# Autodesk Inventor assembly: GA_bilen
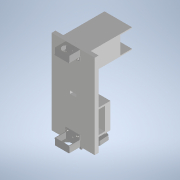
[picture p0: Inventor's stored thumbnail of the model, 180x180]
Saved by Autodesk Inventor 2022.1 (Build 261234020, 234B)
## iProperties
Created: 2022-01-29
Part Number: GA_bilen
Document SubType Name: Assembly
Designer: 46734
Author: 46734
## Documents named in this file (14)
- G:\Min enhet\GA\3d print\GA_bilen.iam
- G:\Min enhet\GA\3d print\Assembly1.iam
- G:\Min enhet\GA\3d print\body.ipt
- G:\Min enhet\GA\3d print\KameraFront v1.ipt
- G:\Min enhet\GA\3d print\poerbankhållare.ipt
- G:\Min enhet\GA\3d print\test hålare.ipt
- G:\Min enhet\GA\3d print\ULTRALJUD GA v2.ipt
- G:\Min enhet\GA\3d print\pir sensor v1.ipt
- G:\Min enhet\GA\3d print\kameraGa Langst ner v1.ipt
- G:\Min enhet\GA\3d print\rpi case 4.ipt
- C:\Users\46734\Documents\Inventor\Content Center Files\R2022\en-US\AS 1420\AS 1420 - 1973 - M3 x 10.ipt
- C:\Users\46734\Documents\Inventor\Content Center Files\R2022\en-US\ANSI B18.3.1M(1)\ANSI B18.3.1M - M2x0,4 x 10(2).ipt
- C:\Users\46734\Documents\Inventor\Content Center Files\R2022\en-US\AS 1420\AS 1420 - 1973 - M4 x 25.ipt
- C:\Users\46734\Documents\Inventor\Content Center Files\R2022\en-US\ANSI B18.2.4.2M\ANSI B18.2.4.2M - M4x0,7 - 7.ipt
## Components (24 placed, 13 different names)
1. Assembly1:1 [sub-assembly] — Mate:1, Flush:1, Flush:2, Insert:1
2. body:1 — Mate:2, Flush:3, Flush:4, Mate:3, Flush:5, Flush:6, Mate:4, Flush:7, Mate:5, Flush:9, Flush:10, Mate:10, Flush:19, Flush:20
3. KameraFront v1:1 — Mate:1, Flush:1, Flush:2
4. poerbankhållare:1 — Mate:2, Flush:3, Flush:4, Rotational:7, Rotational:8, Rotational:9, Rotational:10
5. test hålare:1 — Insert:1, Flush:17, Flush:18, Mate:9, Flush:22, Rotational:11, Rotational:12, Rigid:1, Rotational:13
6. ULTRALJUD GA v2:1 — Mate:5, Flush:9, Flush:10, Rotational:1, Rotational:2
7. pir sensor v1:1 — Mate:4, Flush:7, Flush:8, Rotational:3, Rotational:4
8. pir sensor v1:2 — Mate:3, Flush:5, Flush:6, Flush:8, Rotational:5, Rotational:6
9. kameraGa Langst ner v1:1 — Flush:17, Flush:18, Mate:9, Mate:11, Flush:21
10. rpi case 4:1 — Mate:10, Flush:19, Flush:20, Mate:11, Flush:21, Flush:22
11. AS 1420 - Metric M3 x 10:1 — Rotational:1
12. AS 1420 - Metric M3 x 10:2 — Rotational:4
13. AS 1420 - Metric M3 x 10:3 — Rotational:3
14. AS 1420 - Metric M3 x 10:4 — Rotational:2
15. AS 1420 - Metric M3 x 10:5 — Rotational:6
16. AS 1420 - Metric M3 x 10:6 — Rotational:5
17. AS 1420 - Metric M3 x 10:7 — Rotational:7
18. AS 1420 - Metric M3 x 10:8 — Rotational:8
19. AS 1420 - Metric M3 x 10:9 — Rotational:9
20. AS 1420 - Metric M3 x 10:10 — Rotational:10
21. Broached Socket Head Cap Screw - Metric M2x0,4 x 10:1 — Rotational:12
22. Broached Socket Head Cap Screw - Metric M2x0,4 x 10:2 — Rotational:11
23. AS 1420 - Metric M4 x 25:1 — Rigid:1
24. ANSI B18.2.4.2M M4x0,7:1 — Rotational:13
## Relationships (39: Flush 16, RevoluteJoint 13, Mate 8, Insert 1, WeldJoint 1)
- Mate:1: Assembly1:1 ↔ KameraFront v1:1
- Flush:1: Assembly1:1 ↔ KameraFront v1:1
- Flush:2: Assembly1:1 ↔ KameraFront v1:1
- Insert:1: Assembly1:1 ↔ test hålare:1
- Mate:2: body:1 ↔ poerbankhållare:1
- Flush:3: body:1 ↔ poerbankhållare:1
- Flush:4 (20 mm): body:1 ↔ poerbankhållare:1
- Mate:3: body:1 ↔ pir sensor v1:2
- Flush:5: body:1 ↔ pir sensor v1:2
- Flush:6 (36.5 mm): body:1 ↔ pir sensor v1:2
- Mate:4: body:1 ↔ pir sensor v1:1
- Flush:7: body:1 ↔ pir sensor v1:1
- Flush:8: pir sensor v1:1 ↔ pir sensor v1:2
- Mate:5: body:1 ↔ ULTRALJUD GA v2:1
- Flush:9: body:1 ↔ ULTRALJUD GA v2:1
- Flush:10 (-34.25 mm): body:1 ↔ ULTRALJUD GA v2:1
- Flush:17 (10 mm): test hålare:1 ↔ kameraGa Langst ner v1:1
- Flush:18: test hålare:1 ↔ kameraGa Langst ner v1:1
- Mate:9: test hålare:1 ↔ kameraGa Langst ner v1:1
- Mate:10: body:1 ↔ rpi case 4:1
- Flush:19 (10 mm): body:1 ↔ rpi case 4:1
- Flush:20 (25 mm): body:1 ↔ rpi case 4:1
- Mate:11: kameraGa Langst ner v1:1 ↔ rpi case 4:1
- Flush:21 (30 mm): kameraGa Langst ner v1:1 ↔ rpi case 4:1
- Flush:22 (1.142 mm): test hålare:1 ↔ rpi case 4:1
- Rotational:1 [RevoluteJoint]: ULTRALJUD GA v2:1 ↔ AS 1420 - Metric M3 x 10:1
- Rotational:2 [RevoluteJoint]: ULTRALJUD GA v2:1 ↔ AS 1420 - Metric M3 x 10:4
- Rotational:3 [RevoluteJoint]: pir sensor v1:1 ↔ AS 1420 - Metric M3 x 10:3
- Rotational:4 [RevoluteJoint]: pir sensor v1:1 ↔ AS 1420 - Metric M3 x 10:2
- Rotational:5 [RevoluteJoint]: pir sensor v1:2 ↔ AS 1420 - Metric M3 x 10:6
- Rotational:6 [RevoluteJoint]: pir sensor v1:2 ↔ AS 1420 - Metric M3 x 10:5
- Rotational:7 [RevoluteJoint]: poerbankhållare:1 ↔ AS 1420 - Metric M3 x 10:7
- Rotational:8 [RevoluteJoint]: poerbankhållare:1 ↔ AS 1420 - Metric M3 x 10:8
- Rotational:9 [RevoluteJoint]: poerbankhållare:1 ↔ AS 1420 - Metric M3 x 10:9
- Rotational:10 [RevoluteJoint]: poerbankhållare:1 ↔ AS 1420 - Metric M3 x 10:10
- Rotational:11 [RevoluteJoint]: test hålare:1 ↔ Broached Socket Head Cap Screw - Metric M2x0,4 x 10:2
- Rotational:12 [RevoluteJoint]: test hålare:1 ↔ Broached Socket Head Cap Screw - Metric M2x0,4 x 10:1
- Rigid:1 [WeldJoint]: test hålare:1 ↔ AS 1420 - Metric M4 x 25:1
- Rotational:13 [RevoluteJoint]: test hålare:1 ↔ ANSI B18.2.4.2M M4x0,7:1
